# Autodesk Inventor assembly: face
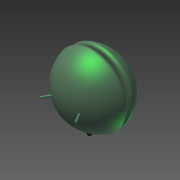
[picture p0: Inventor's stored thumbnail of the model, 180x180]
Saved by Autodesk Inventor 2011 (Build 150239000, 239)
## iProperties
Created: 2013-01-27
Part Number: face
Document SubType Name: Assembly
Designer: bot_m8ker
Author: bot_m8ker
## Documents named in this file (4)
- C:\Users\bot_m8ker\Documents\Inventor\Pac-Droid\face.iam
- C:\Users\bot_m8ker\Documents\Inventor\Pac-Droid\head.ipt
- C:\Users\bot_m8ker\Documents\Inventor\Pac-Droid\eye.ipt
- C:\Users\bot_m8ker\Documents\Inventor\Pac-Droid\bottom.ipt
## Components (4 placed, 3 different names)
1. head:1 — Mate:1, Mate:2, Mate:3, Mate:4
2. eye:1 — Mate:1, Mate:2
3. eye:2 — Mate:3, Mate:4
4. bottom:1 — Mate:9
## Relationships (9: Mate 8, Flush 1)
- Mate:1: head:1 ↔ eye:1
- Mate:2: head:1 ↔ eye:1
- Mate:3: head:1 ↔ eye:2
- Mate:4: head:1 ↔ eye:2
- Flush:1 (10.795 mm)
- Mate:7
- Mate:8
- Mate:9: bottom:1
- Mate:10
